# Autodesk Inventor assembly: Workbench_Frame
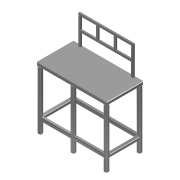
[picture p0: Inventor's stored thumbnail of the model, 180x180]
Saved by Autodesk Inventor 2022 (Build 260148000, 148)
## iProperties
_SolveAssemblyDoc: Frame Generator Solve Assembly
_Version: 15.0.0
Created: 2021-03-15
Part Number: Workbench_Frame
Document SubType Name: Assembly
Designer: jmacmillan
Author: jmacmillan
## Documents named in this file (5)
- C:\Autodesk Inventor 2022 Advanced Assembly Modeling Practice Files\Substitute Model State\Workbench_Frame.iam
- C:\Autodesk Inventor 2022 Advanced Assembly Modeling Practice Files\Substitute Model State\Basic_frame_LowerWorkbench.ipt
- C:\Autodesk Inventor 2022 Advanced Assembly Modeling Practice Files\Substitute Model State\Basic_frame_UpperWorkbench.ipt
- C:\Autodesk Inventor 2022 Advanced Assembly Modeling Practice Files\Substitute Model State\Workbench_Frame\Frame\Frame 1615832763162.iam
- C:\Autodesk Inventor 2022 Advanced Assembly Modeling Practice Files\Substitute Model State\TableTop.ipt
## Components (4 placed, 4 different names)
1. Basic_frame_LowerWorkbench:1 — Mate:3, Mate:4
2. Basic_frame_UpperWorkbench:1 — Mate:3, Mate:4
3. Frame 1615832763162:1 [sub-assembly] — Mate:5, Flush:1, Flush:2
4. TableTop:1 — Mate:5, Flush:1, Flush:2
## Relationships (5: Mate 3, Flush 2)
- Mate:3: Basic_frame_LowerWorkbench:1 ↔ Basic_frame_UpperWorkbench:1
- Mate:4 (245.667 mm): Basic_frame_LowerWorkbench:1 ↔ Basic_frame_UpperWorkbench:1
- Mate:5: Frame 1615832763162:1 ↔ TableTop:1
- Flush:1: Frame 1615832763162:1 ↔ TableTop:1
- Flush:2: Frame 1615832763162:1 ↔ TableTop:1
